# Autodesk Inventor assembly: Elbow Mecha v2
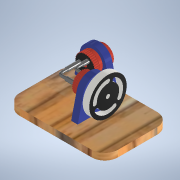
[picture p0: Inventor's stored thumbnail of the model, 180x180]
Saved by Autodesk Inventor 2022 (Build 260153000, 153)
## iProperties
Created: 2022-02-07
Part Number: Elbow Mecha v2
Document SubType Name: Assembly
Designer: joshw
Title: D:/Fab_Labs/Week_3/Fusion/Elbow Mecha v2.step
Sending System: Autodesk Translation Framework v10.13.0.1454
Preprocessor: ST-DEVELOPER v18.1
## Documents named in this file (5)
- D:\Fab_Labs\Week_3\Fusion\Elbow Mecha v2.iam
- D:\Fab_Labs\Week_3\Fusion\Piston.ipt
- D:\Fab_Labs\Week_3\Fusion\Cylinder.ipt
- D:\Fab_Labs\Week_3\Fusion\Component5.ipt
- D:\Fab_Labs\Week_3\Fusion\Component6.ipt
## Components (7 placed, 4 different names)
1. Piston:1 — Cylindrical:5, Cylindrical:6
2. Piston:2 — Cylindrical:3, Cylindrical:4
3. Piston:3 — Cylindrical:1, Cylindrical:2
4. Cylinder:1 — Rotational:2, Cylindrical:1, Cylindrical:4, Cylindrical:6, Rigid:1, Angle:1
5. Cylinder:2 — Rotational:1, Cylindrical:2, Cylindrical:3, Cylindrical:5
6. Component5:1 — Rotational:1, Rotational:2
7. Component6:1 — Rigid:1
## Relationships (10: CylindricalJoint 6, RevoluteJoint 2, WeldJoint 1, Angle 1)
- Rotational:1 [RevoluteJoint]: Cylinder:2 ↔ Component5:1
- Rotational:2 [RevoluteJoint]: Cylinder:1 ↔ Component5:1
- Cylindrical:1: Piston:3 ↔ Cylinder:1
- Cylindrical:2: Piston:3 ↔ Cylinder:2
- Cylindrical:3: Piston:2 ↔ Cylinder:2
- Cylindrical:4: Piston:2 ↔ Cylinder:1
- Cylindrical:5: Piston:1 ↔ Cylinder:2
- Cylindrical:6: Piston:1 ↔ Cylinder:1
- Rigid:1 [WeldJoint]: Cylinder:1 ↔ Component6:1
- Angle:1 (0 deg): Cylinder:1
